# Autodesk Inventor assembly: ASY HPR 290 Support Frame
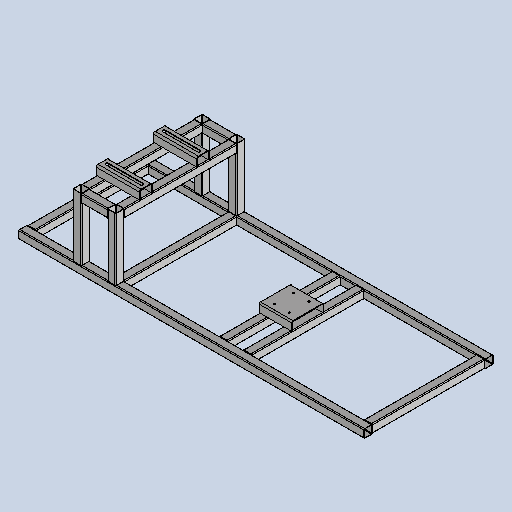
[picture p0: Inventor's stored thumbnail of the model, 512x512]
Saved by Autodesk Inventor 2025.1 (Build 291241020, 241B)
## iProperties
Created: 2025-02-25
Part Number: ASY HPR 290 Support Frame
Document SubType Name: Assembly
Designer: user
Author: user
## Documents named in this file (4)
- C:\Users\user\YandexDisk-badmisterfox\home pc\Inventor\NDM-VOS_powder_hopper\ASY HPR 290 Support Frame.iam
- C:\Users\user\YandexDisk-badmisterfox\home pc\Inventor\NDM-VOS_powder_hopper\ASY Augur motor frame 500.iam
- C:\Users\user\YandexDisk-badmisterfox\home pc\Inventor\NDM-VOS_powder_hopper\NDM-VOS 715 flange.ipt
- C:\Users\user\YandexDisk-badmisterfox\home pc\Inventor\NDM-VOS_powder_hopper\FL3.6.2  Motor pillar.ipt
## Components (4 placed, 3 different names)
1. ASY Augur motor frame 500:1 [sub-assembly]
2. NDM-VOS 715 flange:1
3. FL3.6.2  Motor pillar:1
4. NDM-VOS 715 flange:2
## Relationships (7: Mate 4, Flush 3)
- [Mate]: ASY Augur motor frame 500:1 ↔ NDM-VOS 715 flange:1
- [Flush]: ASY Augur motor frame 500:1 ↔ NDM-VOS 715 flange:1
- [Mate]: ASY Augur motor frame 500:1 ↔ FL3.6.2  Motor pillar:1
- [Flush]: ASY Augur motor frame 500:1 ↔ FL3.6.2  Motor pillar:1
- [Mate]: ASY Augur motor frame 500:1 ↔ FL3.6.2  Motor pillar:1
- [Mate]: ASY Augur motor frame 500:1 ↔ NDM-VOS 715 flange:2
- [Flush]: ASY Augur motor frame 500:1 ↔ NDM-VOS 715 flange:2
